# Autodesk Inventor assembly: frame_bottom
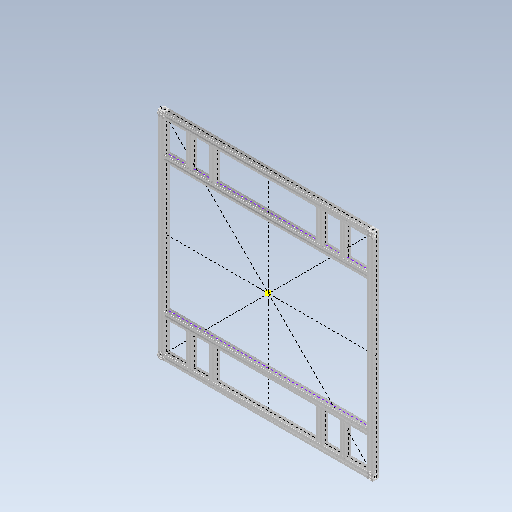
[picture p0: Inventor's stored thumbnail of the model, 512x512]
Saved by Autodesk Inventor 2021.3 (Build 253353000, 353)
## iProperties
_SolveAssemblyDoc: Frame Generator Solve Assembly
_Version: 15.0.0
Created: 2023-04-06
Part Number: frame_bottom
Document SubType Name: Assembly
Designer: nxf77172
Author: nxf77172
## Documents named in this file (4)
- C:\Users\nxf77172\Desktop\mechanical_cleaned\custom_parts\frame\frame_bottom.iam
- C:\Users\nxf77172\Desktop\mechanical_cleaned\custom_parts\frame\frame_outline.ipt
- C:\Users\nxf77172\Desktop\mechanical_cleaned\custom_parts\frame\frame_bottom\Frame\Frame 1680795495162.iam
- C:\Users\nxf77172\Desktop\mechanical_cleaned\custom_parts\aluminium profile\angle_connector_x3.ipt
## Components (6 placed, 3 different names)
1. frame_outline:1 — Mate:1, Mate:2
2. Frame 1680795495162:1 [sub-assembly] — Insert:1, Angle:1, Angle:3, Insert:2, Angle:4, Insert:3, Angle:5, Insert:4
3. angle_connector_x3:1 — Insert:1, Angle:1
4. angle_connector_x3:2 — Angle:3, Insert:2
5. angle_connector_x3:3 — Angle:4, Insert:3
6. angle_connector_x3:4 — Angle:5, Insert:4
## Relationships (10: Insert 4, Angle 4, Mate 2)
- Mate:1: frame_outline:1
- Mate:2: frame_outline:1
- Insert:1: Frame 1680795495162:1 ↔ angle_connector_x3:1
- Angle:1 (0 deg): Frame 1680795495162:1 ↔ angle_connector_x3:1
- Angle:3 (180 deg): Frame 1680795495162:1 ↔ angle_connector_x3:2
- Insert:2: Frame 1680795495162:1 ↔ angle_connector_x3:2
- Angle:4 (0 deg): Frame 1680795495162:1 ↔ angle_connector_x3:3
- Insert:3: Frame 1680795495162:1 ↔ angle_connector_x3:3
- Angle:5 (180 deg): Frame 1680795495162:1 ↔ angle_connector_x3:4
- Insert:4: Frame 1680795495162:1 ↔ angle_connector_x3:4
